# Autodesk Inventor assembly: Сборка
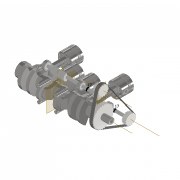
[picture p0: Inventor's stored thumbnail of the model, 180x180]
Saved by Autodesk Inventor 2021 (Build 250183000, 183)
## iProperties
Created: 2021-06-15
Part Number: Сборка
Document SubType Name: Assembly
Designer: panda
Mass: 39332.9 g
Surface Area: 9886.22 cm^2
Volume: 5300.69 cm^3
Density: 7.42033 g/cm^3
Author: panda
## Documents named in this file (6)
- C:\Users\panda\Desktop\vkrb\сборка\Сборка.iam
- C:\Users\panda\Desktop\vkrb\сборка\поршень_шатун_палец.iam
- C:\Users\panda\Desktop\vkrb\сборка\crankshaft.ipt
- C:\Users\panda\Desktop\vkrb\сборка\сборка_балансирного_вала.iam
- C:\Users\panda\Desktop\vkrb\сборка\Сборка\Мастер проектирования\Цилиндрическое зубчатое зацепление2.iam
- C:\Users\panda\Desktop\vkrb\сборка\Сборка\Мастер проектирования\Передача с помощью зубчатых ремней9.iam
## Components (9 placed, 5 different names)
1. поршень_шатун_палец:2 [sub-assembly] — Совмещение:4, Угол:2
2. поршень_шатун_палец:4 [sub-assembly] — Совмещение:3, Угол:3, Угол:4
3. поршень_шатун_палец:5 [sub-assembly] — Совмещение:2, Угол:4
4. crankshaft:1 — Совмещение:2, Совмещение:3, Совмещение:4, Совмещение:5, Угол:1, Совмещение:6, Совмещение:7, Заподлицо:1, Совмещение:8, Совмещение:10, Совмещение:11, Заподлицо:3, Совмещение:12, Совмещение:16, Заподлицо:5
5. поршень_шатун_палец:6 [sub-assembly] — Совмещение:5, Угол:1, Угол:2, Угол:3
6. сборка_балансирного_вала:2 [sub-assembly] — Совмещение:8, Совмещение:9, Угол:5, Заподлицо:2, Совмещение:12, Совмещение:13, Совмещение:14, Совмещение:15
7. сборка_балансирного_вала:3 [sub-assembly] — Угол:5, Совмещение:10, Совмещение:11, Заподлицо:2
8. Цилиндрическое зубчатое зацепление:1 [sub-assembly] — Совмещение:13, Совмещение:14, Совмещение:15, Заподлицо:4
9. Передача с помощью зубчатых ремней:1 [sub-assembly]
## Relationships (25: Mate 15, Angle 5, Flush 5)
- Совмещение:2 [Mate]: поршень_шатун_палец:5 ↔ crankshaft:1
- Совмещение:3 [Mate]: поршень_шатун_палец:4 ↔ crankshaft:1
- Совмещение:4 [Mate]: поршень_шатун_палец:2 ↔ crankshaft:1
- Совмещение:5 [Mate]: crankshaft:1 ↔ поршень_шатун_палец:6
- Угол:1 [Angle] (180 deg): crankshaft:1 ↔ поршень_шатун_палец:6
- Угол:2 [Angle] (0 deg): поршень_шатун_палец:2 ↔ поршень_шатун_палец:6
- Совмещение:6 [Mate]: crankshaft:1
- Угол:3 [Angle] (0 deg): поршень_шатун_палец:4 ↔ поршень_шатун_палец:6
- Угол:4 [Angle] (0 deg): поршень_шатун_палец:4 ↔ поршень_шатун_палец:5
- Совмещение:7 [Mate]: crankshaft:1
- Заподлицо:1 [Flush]: crankshaft:1
- Совмещение:8 [Mate] (100 mm): crankshaft:1 ↔ сборка_балансирного_вала:2
- Совмещение:9 [Mate]: сборка_балансирного_вала:2
- Угол:5 [Angle] (0 deg): сборка_балансирного_вала:2 ↔ сборка_балансирного_вала:3
- Совмещение:10 [Mate] (-170 mm): crankshaft:1 ↔ сборка_балансирного_вала:3
- Совмещение:11 [Mate] (-100 mm): crankshaft:1 ↔ сборка_балансирного_вала:3
- Заподлицо:2 [Flush]: сборка_балансирного_вала:2 ↔ сборка_балансирного_вала:3
- Заподлицо:3 [Flush] (9.017 mm): crankshaft:1
- Совмещение:12 [Mate]: crankshaft:1 ↔ сборка_балансирного_вала:2
- Совмещение:13 [Mate]: сборка_балансирного_вала:2 ↔ Цилиндрическое зубчатое зацепление:1
- Совмещение:14 [Mate]: сборка_балансирного_вала:2 ↔ Цилиндрическое зубчатое зацепление:1
- Совмещение:15 [Mate]: сборка_балансирного_вала:2 ↔ Цилиндрическое зубчатое зацепление:1
- Заподлицо:4 [Flush] (12.446 mm): Цилиндрическое зубчатое зацепление:1
- Совмещение:16 [Mate]: crankshaft:1
- Заподлицо:5 [Flush] (16 mm): crankshaft:1
